# Autodesk Inventor assembly: MG-Rolle
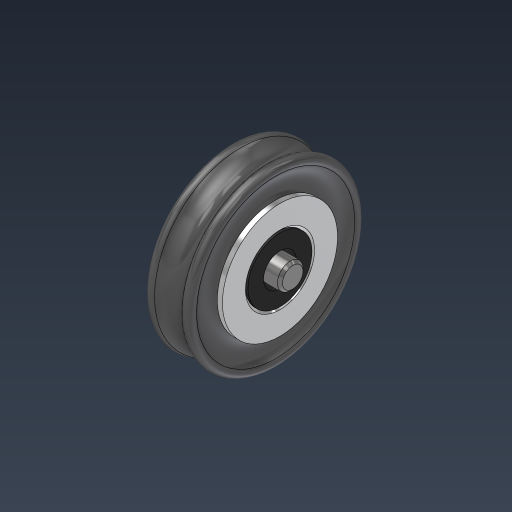
[picture p0: Inventor's stored thumbnail of the model, 512x512]
Saved by Autodesk Inventor 2023.1 (Build 271208000, 208)
## iProperties
Part Number: MG-Rolle
Material: Generisch
Document SubType Name: Assembly
Designer: rYan
Mass: 1.3472 g
Surface Area: 13.7675 cm^2
Volume: 0.879852 cm^3
Density: 1.53117 g/cm^3
Author: rYan
## Documents named in this file (5)
- D:\TIGERsGIT\Hardware\mechanik\2024\Inventor\Robot\Drive Train\Common\MG-Rolle.iam
- D:\TIGERsGIT\Hardware\mechanik\2024\Inventor\Robot\Drive Train\Common\Rolle.ipt
- D:\TIGERsGIT\Hardware\mechanik\2024\Inventor\Purchased Parts\X-Ring 5.94x3.53.ipt
- D:\TIGERsGIT\Hardware\mechanik\2024\Inventor\Purchased Parts\Gleitlager MSM-0205-02.ipt
- D:\TIGERsGIT\Hardware\mechanik\2024\Inventor\Robot\Drive Train\Common\Welle Querrolle Quad.ipt
## Components (5 placed, 4 different names)
1. X-Ring 5.94x3.53:1 — Passend:7, Fluchtend:2
2. Rolle:1 — Passend:12, Passend:13, Einfügen:1, Einfügen:2, Einfügen:3
3. Gleitlager MSM-0205-02:1 — Einfügen:1
4. Gleitlager MSM-0205-02:2 — Einfügen:2
5. Welle Querrolle Quad:1 — Einfügen:3
## Relationships (8: Mate 3, Insert 3, Flush 2)
- Passend:7 [Mate]: X-Ring 5.94x3.53:1
- Fluchtend:2 [Flush]: X-Ring 5.94x3.53:1
- Fluchtend:4 [Flush] (-6.8 mm)
- Passend:12 [Mate]: Rolle:1
- Passend:13 [Mate]: Rolle:1
- Einfügen:1 [Insert]: Rolle:1 ↔ Gleitlager MSM-0205-02:1
- Einfügen:2 [Insert]: Rolle:1 ↔ Gleitlager MSM-0205-02:2
- Einfügen:3 [Insert] (0.1 mm): Rolle:1 ↔ Welle Querrolle Quad:1
